# Autodesk Inventor assembly: Camera_Full
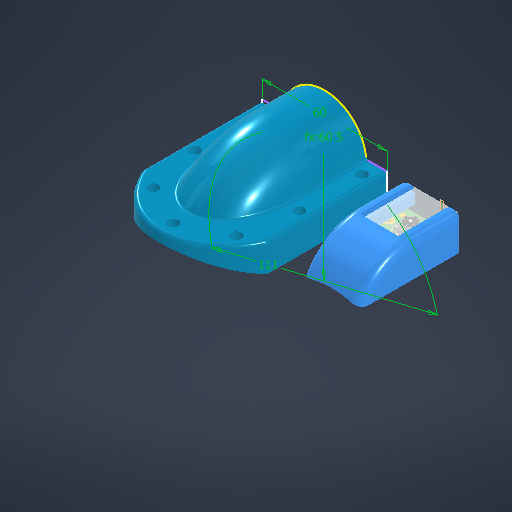
[picture p0: Inventor's stored thumbnail of the model, 512x512]
Saved by Autodesk Inventor 2025.2 (Build 292293000, 293)
## iProperties
Created: 2025-06-17
Part Number: Camera_Full
Document SubType Name: Assembly
Designer: user
Author: user
## Documents named in this file (5)
- E:\nakuu\Repo\repoo\nakuja_bruh\GLENN\Camera mold\camera Full\Camera_Full.iam
- E:\nakuu\Repo\repoo\nakuja_bruh\GLENN\Camera mold\camera Full\Camera.ipt
- E:\nakuu\Repo\repoo\nakuja_bruh\GLENN\Camera mold\camera Full\Cam V2.1 v1.ipt
- E:\nakuu\Repo\repoo\nakuja_bruh\GLENN\Camera mold\camera Full\Cover.ipt
- E:\nakuu\Repo\repoo\nakuja_bruh\GLENN\Camera mold\Down facing camera.ipt
## Components (5 placed, 4 different names)
1. Camera:1 — Mate:1
2. Cam V2.1 v1:1
3. Cover:1 — Mate:1
4. Down facing camera:1 — Mate:2
5. Cam V2.1 v1:2 — Mate:2
## Relationships (2: Mate 2)
- Mate:1: Camera:1 ↔ Cover:1
- Mate:2: Down facing camera:1 ↔ Cam V2.1 v1:2
